# Autodesk Inventor assembly: HEAD
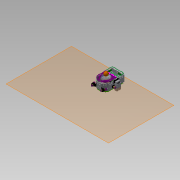
[picture p0: Inventor's stored thumbnail of the model, 180x180]
Saved by Autodesk Inventor 2015 SP1 (Build 190203100, 203)
## iProperties
Created: 2015-02-03
Part Number: HEAD
Document SubType Name: Assembly
Designer: Rafi Kurnia Putra
Author: Rafi Kurnia Putra
## Documents named in this file (23)
- D:\Dropbox\krpai berkaki trui 2015\ROBUSTA\MEKANIK\ROBUSTA\Assembly Kepala.iam
- D:\Dropbox\krpai berkaki trui 2015\ROBUSTA\MEKANIK\ROBUSTA\Assembly STM32 + SHIELD.iam
- D:\Dropbox\krpai berkaki trui 2015\ROBUSTA\MEKANIK\ROBUSTA\Spacer 2cm.ipt
- D:\Dropbox\krpai berkaki trui 2015\ROBUSTA\MEKANIK\ROBUSTA\Sound Detect V2.ipt
- D:\Dropbox\krpai berkaki trui 2015\ROBUSTA\MEKANIK\ROBUSTA\Assembly RPLIDAR.iam
- D:\Dropbox\krpai berkaki trui 2015\ROBUSTA\MEKANIK\ROBUSTA\Proximity.ipt
- D:\Dropbox\krpai berkaki trui 2015\ROBUSTA\MEKANIK\ROBUSTA\Proximity Gear.ipt
- D:\Dropbox\krpai berkaki trui 2015\ROBUSTA\MEKANIK\ROBUSTA\Power Distribution V2.ipt
- D:\Dropbox\krpai berkaki trui 2015\ROBUSTA\MEKANIK\ROBUSTA\I2C.ipt
- D:\Dropbox\krpai berkaki trui 2015\ROBUSTA\MEKANIK\ROBUSTA\Bola Pingpong.ipt
- D:\Dropbox\krpai berkaki trui 2015\ROBUSTA\MEKANIK\ROBUSTA\Kepala Tutup.ipt
- D:\Dropbox\krpai berkaki trui 2015\ROBUSTA\MEKANIK\ROBUSTA\Start Stop.ipt
- D:\Dropbox\krpai berkaki trui 2015\ROBUSTA\MEKANIK\ROBUSTA\Assembly Proximity V3.iam
- D:\Dropbox\krpai berkaki trui 2015\ROBUSTA\MEKANIK\ROBUSTA\Spacer 1cm.ipt
- D:\Dropbox\krpai berkaki trui 2015\ROBUSTA\MEKANIK\ROBUSTA\Plat.ipt
- D:\Dropbox\krpai berkaki trui 2015\ROBUSTA\MEKANIK\ROBUSTA\Baterai 1.0.ipt
- D:\Dropbox\krpai berkaki trui 2015\ROBUSTA\MEKANIK\ROBUSTA\Baterai 1.3.ipt
- D:\Dropbox\krpai berkaki trui 2015\ROBUSTA\MEKANIK\ROBUSTA\Cover Baterai.ipt
- D:\Dropbox\krpai berkaki trui 2015\ROBUSTA\MEKANIK\ROBUSTA\Kepala Depan 2.ipt
- D:\Dropbox\krpai berkaki trui 2015\ROBUSTA\MEKANIK\ROBUSTA\srf10.ipt
- D:\Dropbox\krpai berkaki trui 2015\ROBUSTA\MEKANIK\ROBUSTA\Kepala Tengah 2.ipt
- D:\Dropbox\krpai berkaki trui 2015\ROBUSTA\MEKANIK\ROBUSTA\Cover Batera 3i.ipt
- D:\Dropbox\krpai berkaki trui 2015\ROBUSTA\MEKANIK\ROBUSTA\Kepala Belakang 2.ipt
## Components (56 placed, 22 different names)
1. srf10:3 — Mate:191, Mate:192, Mate:193
2. srf10:4 — Mate:185, Mate:186, Mate:187
3. srf10:5 — Mate:197, Mate:198, Mate:199
4. srf10:1 — Mate:194, Mate:195, Mate:196
5. srf10:2 — Mate:188, Mate:189, Mate:190
6. Kepala Depan 2:1 — Mate:1, Flush:2, Flush:3, Mate:29, Mate:36, Mate:57, Mate:62, Flush:35, Mate:110, Mate:112, Mate:114, Mate:115, Mate:149, Tangent:12, Tangent:13, Mate:150, Tangent:14, Tangent:15, Angle:2, Mate:151, Tangent:17, Angle:3, Tangent:18, Mate:162, Mate:163, Mate:172, Mate:176, Mate:185, Mate:186, Mate:187, Mate:188, Mate:189, Mate:190, Mate:191, Mate:192, Mate:193, Mate:194, Mate:195, Mate:196, Mate:197, Mate:198, Mate:199
7. Assembly STM32 + SHIELD:1 [sub-assembly] — Mate:21, Mate:22, Mate:23, Mate:24, Mate:25, Mate:26, Mate:27, Mate:28, Mate:44, Mate:69, Tangent:1, Mate:107
8. Spacer 2cm:1 — Mate:21, Mate:25
9. Spacer 2cm:2 — Mate:22, Mate:26
10. Spacer 2cm:3 — Mate:24, Mate:28, Mate:84
11. Spacer 2cm:4 — Mate:23, Mate:27
12. Kepala Tengah 2:1 — Flush:2, Flush:3, Mate:29, Flush:10, Mate:43, Flush:18, Mate:63, Mate:64, Tangent:2, Mate:75, Mate:77, Mate:81, Mate:83, Mate:142, Mate:145, Mate:146, Mate:147, Mate:168, Mate:169, Mate:171, Mate:173, Mate:174, Mate:175, Mate:177, Mate:178, Flush:41, Flush:42, Mate:180, Mate:181, Mate:182, Flush:45, Mate:200, Mate:201
13. Sound Detect V2:1 — Mate:36, Mate:63, Mate:64
14. Assembly RPLIDAR:1 [sub-assembly] — Flush:4, Mate:38, Mate:39, Mate:40, Mate:41, Flush:5, Flush:6, Flush:7, Flush:8, Tangent:1, Tangent:7, Mate:154, Mate:155, Mate:210
15. Spacer 2cm:5 — Mate:38, Flush:7, Mate:62
16. Spacer 2cm:6 — Mate:41, Flush:5
17. Spacer 2cm:7 — Mate:39, Flush:6
18. Spacer 2cm:8 — Mate:40, Flush:8
19. Kepala Belakang 2:1 — Flush:9, Flush:10, Mate:43, Mate:69, Mate:84, Mate:94, Angle:1, Mate:111, Mate:113, Mate:116, Mate:117, Mate:131, Mate:170, Mate:179, Flush:46, Mate:202, Mate:203, Mate:204, Mate:205, Mate:206, Mate:207, Mate:208, Mate:209
20. srf10:6 — Mate:205, Mate:206, Mate:207
21. srf10:7 — Mate:202, Mate:203, Mate:204
22. Proximity:1 — Tangent:2, Mate:76, Mate:78, Flush:24, Tangent:12, Flush:41
23. Proximity Gear:1 — Mate:75, Mate:76
24. Proximity Gear:2 — Mate:77, Mate:78
25. Proximity:2 — Flush:24, Mate:80, Mate:82, Tangent:13, Flush:42
26. Proximity Gear:3 — Mate:80, Mate:81
27. Proximity Gear:4 — Mate:82, Mate:83
28. Power Distribution V2:1 — Mate:94, Angle:1, Mate:95, Mate:131
29. I2C:1 — Mate:99, Flush:35, Mate:118
30. Bola Pingpong:1 — Tangent:7, Mate:101, Mate:154, Mate:155
31. Kepala Tutup:1 — Flush:37, Mate:106
32. Start Stop:1 — Mate:106, Mate:107
33. Assembly Proximity V3:1 [sub-assembly] — Mate:150, Tangent:14, Tangent:15, Angle:2
34. Assembly Proximity V3:2 [sub-assembly] — Mate:151, Tangent:17, Angle:3, Tangent:18
35. Spacer 1cm:1 — Mate:112, Mate:115, Mate:118
36. Spacer 1cm:2 — Mate:113, Mate:117
37. Spacer 1cm:3 — Mate:111, Mate:116
38. Spacer 1cm:4 — Mate:110, Mate:114
39. Spacer 2cm:15 — Mate:132, Mate:133
40. Spacer 2cm:9 — Mate:132, Mate:133, Mate:149
41. Spacer 2cm:16
42. Spacer 2cm:10 — Mate:142, Mate:146
43. Spacer 2cm:14 — Mate:162, Mate:163, Mate:164, Mate:165
44. Spacer 2cm:13 — Mate:143, Mate:144
45. Spacer 2cm:12 — Mate:143, Mate:144, Mate:145, Mate:147
46. Spacer 2cm:17 — Mate:164, Mate:165
47. srf10:8 — Mate:208, Mate:209
48. Plat:1 — Mate:168, Mate:169, Mate:170
49. Plat:2 — Mate:171, Mate:172, Mate:173
50. Plat:3 — Mate:174, Mate:176, Mate:177
51. Plat:4 — Mate:175, Mate:178, Mate:179
52. Baterai 1.0:1 — Mate:180, Flush:43, Flush:44, Mate:183, Mate:184
53. Baterai 1.3:1 — Mate:181, Flush:43, Flush:44
54. Cover Baterai:1 — Mate:182, Flush:45, Flush:46, Mate:183, Mate:184
55. Cover Batera 3i:1 — Mate:200, Mate:201
56. Kepala Tutup:2 — Mate:210
## Relationships (142: Mate 110, Flush 20, Tangent 9, Angle 3)
- Mate:1: Kepala Depan 2:1
- Mate:21: Assembly STM32 + SHIELD:1 ↔ Spacer 2cm:1
- Mate:22: Assembly STM32 + SHIELD:1 ↔ Spacer 2cm:2
- Mate:23: Assembly STM32 + SHIELD:1 ↔ Spacer 2cm:4
- Mate:24: Assembly STM32 + SHIELD:1 ↔ Spacer 2cm:3
- Mate:25: Assembly STM32 + SHIELD:1 ↔ Spacer 2cm:1
- Mate:26: Assembly STM32 + SHIELD:1 ↔ Spacer 2cm:2
- Mate:27: Assembly STM32 + SHIELD:1 ↔ Spacer 2cm:4
- Mate:28: Assembly STM32 + SHIELD:1 ↔ Spacer 2cm:3
- Flush:2: Kepala Depan 2:1 ↔ Kepala Tengah 2:1
- Flush:3: Kepala Depan 2:1 ↔ Kepala Tengah 2:1
- Mate:29: Kepala Depan 2:1 ↔ Kepala Tengah 2:1
- Mate:36: Kepala Depan 2:1 ↔ Sound Detect V2:1
- Flush:4: Assembly RPLIDAR:1
- Mate:38: Assembly RPLIDAR:1 ↔ Spacer 2cm:5
- Mate:39: Assembly RPLIDAR:1 ↔ Spacer 2cm:7
- Mate:40: Assembly RPLIDAR:1 ↔ Spacer 2cm:8
- Mate:41: Assembly RPLIDAR:1 ↔ Spacer 2cm:6
- Flush:5: Assembly RPLIDAR:1 ↔ Spacer 2cm:6
- Flush:6: Assembly RPLIDAR:1 ↔ Spacer 2cm:7
- Flush:7: Assembly RPLIDAR:1 ↔ Spacer 2cm:5
- Flush:8: Assembly RPLIDAR:1 ↔ Spacer 2cm:8
- Flush:9: Kepala Belakang 2:1
- Flush:10: Kepala Tengah 2:1 ↔ Kepala Belakang 2:1
- Mate:43: Kepala Tengah 2:1 ↔ Kepala Belakang 2:1
- Mate:44: Assembly STM32 + SHIELD:1
- Mate:57: Kepala Depan 2:1
- Flush:18: Kepala Tengah 2:1
- Mate:62: Kepala Depan 2:1 ↔ Spacer 2cm:5
- Mate:63 (15 mm): Kepala Tengah 2:1 ↔ Sound Detect V2:1
- Mate:64 (10 mm): Kepala Tengah 2:1 ↔ Sound Detect V2:1
- Mate:69 (3.31 mm): Assembly STM32 + SHIELD:1 ↔ Kepala Belakang 2:1
- Tangent:1 (15 mm): Assembly STM32 + SHIELD:1 ↔ Assembly RPLIDAR:1
- Tangent:2 (5 mm): Kepala Tengah 2:1 ↔ Proximity:1
- Mate:75: Kepala Tengah 2:1 ↔ Proximity Gear:1
- Mate:76: Proximity:1 ↔ Proximity Gear:1
- Mate:77: Kepala Tengah 2:1 ↔ Proximity Gear:2
- Mate:78: Proximity:1 ↔ Proximity Gear:2
- Flush:24: Proximity:1 ↔ Proximity:2
- Mate:80: Proximity:2 ↔ Proximity Gear:3
- Mate:81: Kepala Tengah 2:1 ↔ Proximity Gear:3
- Mate:82: Proximity:2 ↔ Proximity Gear:4
- Mate:83: Kepala Tengah 2:1 ↔ Proximity Gear:4
- Mate:84: Spacer 2cm:3 ↔ Kepala Belakang 2:1
- Mate:94: Kepala Belakang 2:1 ↔ Power Distribution V2:1
- Angle:1 (0 deg): Kepala Belakang 2:1 ↔ Power Distribution V2:1
- Mate:95: Power Distribution V2:1
- Mate:99: I2C:1
- Flush:35 (5.2 mm): Kepala Depan 2:1 ↔ I2C:1
- Tangent:7: Assembly RPLIDAR:1 ↔ Bola Pingpong:1
- Mate:101: Bola Pingpong:1
- Flush:37: Kepala Tutup:1
- Mate:106: Kepala Tutup:1 ↔ Start Stop:1
- Mate:107: Assembly STM32 + SHIELD:1 ↔ Start Stop:1
- Mate:110: Kepala Depan 2:1 ↔ Spacer 1cm:4
- Mate:111: Kepala Belakang 2:1 ↔ Spacer 1cm:3
- Mate:112: Kepala Depan 2:1 ↔ Spacer 1cm:1
- Mate:113: Kepala Belakang 2:1 ↔ Spacer 1cm:2
- Mate:114: Kepala Depan 2:1 ↔ Spacer 1cm:4
- Mate:115: Kepala Depan 2:1 ↔ Spacer 1cm:1
- Mate:116: Kepala Belakang 2:1 ↔ Spacer 1cm:3
- Mate:117: Kepala Belakang 2:1 ↔ Spacer 1cm:2
- Mate:118: I2C:1 ↔ Spacer 1cm:1
- Mate:131: Kepala Belakang 2:1 ↔ Power Distribution V2:1
- Mate:132: Spacer 2cm:15 ↔ Spacer 2cm:9
- Mate:133: Spacer 2cm:15 ↔ Spacer 2cm:9
- [Mate]: Spacer 2cm:16 ↔ Spacer 2cm:10
- [Mate]: Spacer 2cm:16 ↔ Spacer 2cm:10
- Mate:142: Kepala Tengah 2:1 ↔ Spacer 2cm:10
- Mate:143: Spacer 2cm:13 ↔ Spacer 2cm:12
- Mate:144: Spacer 2cm:13 ↔ Spacer 2cm:12
- Mate:145: Kepala Tengah 2:1 ↔ Spacer 2cm:12
- Mate:146: Kepala Tengah 2:1 ↔ Spacer 2cm:10
- Mate:147: Kepala Tengah 2:1 ↔ Spacer 2cm:12
- Mate:149: Kepala Depan 2:1 ↔ Spacer 2cm:9
- Tangent:12 (37.5 mm): Kepala Depan 2:1 ↔ Proximity:1
- Tangent:13 (37.5 mm): Kepala Depan 2:1 ↔ Proximity:2
- Mate:150: Kepala Depan 2:1 ↔ Assembly Proximity V3:1
- Tangent:14 (13.5 mm): Kepala Depan 2:1 ↔ Assembly Proximity V3:1
- Tangent:15 (40 mm): Kepala Depan 2:1 ↔ Assembly Proximity V3:1
- Angle:2 (0 deg): Kepala Depan 2:1 ↔ Assembly Proximity V3:1
- Mate:151: Kepala Depan 2:1 ↔ Assembly Proximity V3:2
- Tangent:17 (40 mm): Kepala Depan 2:1 ↔ Assembly Proximity V3:2
- Angle:3 (0 deg): Kepala Depan 2:1 ↔ Assembly Proximity V3:2
- Tangent:18 (13.5 mm): Kepala Depan 2:1 ↔ Assembly Proximity V3:2
- Mate:154: Assembly RPLIDAR:1 ↔ Bola Pingpong:1
- Mate:155: Assembly RPLIDAR:1 ↔ Bola Pingpong:1
- Mate:162: Kepala Depan 2:1 ↔ Spacer 2cm:14
- Mate:163: Kepala Depan 2:1 ↔ Spacer 2cm:14
- Mate:164: Spacer 2cm:14 ↔ Spacer 2cm:17
- Mate:165: Spacer 2cm:14 ↔ Spacer 2cm:17
- [Mate]: srf10:8
- Mate:168: Kepala Tengah 2:1 ↔ Plat:1
- Mate:169: Kepala Tengah 2:1 ↔ Plat:1
- Mate:170: Kepala Belakang 2:1 ↔ Plat:1
- Mate:171: Kepala Tengah 2:1 ↔ Plat:2
- Mate:172: Kepala Depan 2:1 ↔ Plat:2
- Mate:173: Kepala Tengah 2:1 ↔ Plat:2
- Mate:174: Kepala Tengah 2:1 ↔ Plat:3
- Mate:175: Kepala Tengah 2:1 ↔ Plat:4
- Mate:176: Kepala Depan 2:1 ↔ Plat:3
- Mate:177: Kepala Tengah 2:1 ↔ Plat:3
- Mate:178: Kepala Tengah 2:1 ↔ Plat:4
- Mate:179: Kepala Belakang 2:1 ↔ Plat:4
- Flush:41 (-25 mm): Kepala Tengah 2:1 ↔ Proximity:1
- Flush:42 (-25 mm): Kepala Tengah 2:1 ↔ Proximity:2
- Mate:180: Kepala Tengah 2:1 ↔ Baterai 1.0:1
- Mate:181: Kepala Tengah 2:1 ↔ Baterai 1.3:1
- Flush:43: Baterai 1.0:1 ↔ Baterai 1.3:1
- Flush:44: Baterai 1.0:1 ↔ Baterai 1.3:1
- Mate:182: Kepala Tengah 2:1 ↔ Cover Baterai:1
- Flush:45: Kepala Tengah 2:1 ↔ Cover Baterai:1
- Flush:46: Kepala Belakang 2:1 ↔ Cover Baterai:1
- Mate:183: Baterai 1.0:1 ↔ Cover Baterai:1
- Mate:184 (0.25 mm): Baterai 1.0:1 ↔ Cover Baterai:1
- Mate:185: srf10:4 ↔ Kepala Depan 2:1
- Mate:186: srf10:4 ↔ Kepala Depan 2:1
- Mate:187: srf10:4 ↔ Kepala Depan 2:1
- Mate:188: srf10:2 ↔ Kepala Depan 2:1
- Mate:189: srf10:2 ↔ Kepala Depan 2:1
- Mate:190: srf10:2 ↔ Kepala Depan 2:1
- Mate:191: srf10:3 ↔ Kepala Depan 2:1
- Mate:192: srf10:3 ↔ Kepala Depan 2:1
- Mate:193: srf10:3 ↔ Kepala Depan 2:1
- Mate:194: srf10:1 ↔ Kepala Depan 2:1
- Mate:195: srf10:1 ↔ Kepala Depan 2:1
- Mate:196: srf10:1 ↔ Kepala Depan 2:1
- Mate:197: srf10:5 ↔ Kepala Depan 2:1
- Mate:198: srf10:5 ↔ Kepala Depan 2:1
- Mate:199: srf10:5 ↔ Kepala Depan 2:1
- Mate:200: Kepala Tengah 2:1 ↔ Cover Batera 3i:1
- Mate:201: Kepala Tengah 2:1 ↔ Cover Batera 3i:1
- Mate:202: Kepala Belakang 2:1 ↔ srf10:7
- Mate:203: Kepala Belakang 2:1 ↔ srf10:7
- Mate:204: Kepala Belakang 2:1 ↔ srf10:7
- Mate:205: Kepala Belakang 2:1 ↔ srf10:6
- Mate:206: Kepala Belakang 2:1 ↔ srf10:6
- Mate:207: Kepala Belakang 2:1 ↔ srf10:6
- Mate:208: Kepala Belakang 2:1 ↔ srf10:8
- Mate:209: Kepala Belakang 2:1 ↔ srf10:8
- Mate:210: Assembly RPLIDAR:1 ↔ Kepala Tutup:2
- Flush:47 (75.5 mm)
## Named parameters: d515_d513 = 0 mm, d516_d514 = 0 mm
